# Autodesk Inventor assembly: Vise
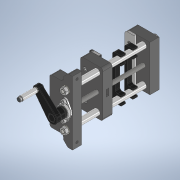
[picture p0: Inventor's stored thumbnail of the model, 180x180]
Saved by Autodesk Inventor 2020.2 (Build 242310000, 310)
## iProperties
Created: 2021-06-22
Part Number: Vise
Document SubType Name: Assembly
Designer: JK
Author: JK
## Documents named in this file (24)
- C:\Users\JK\Documents\Inventor\Vise\Vise.iam
- C:\Users\JK\Documents\Inventor\Vise\Mobile Jaw.ipt
- C:\Users\JK\Documents\Inventor\Vise\Stationary Jaw.ipt
- C:\Users\JK\Documents\Inventor\Vise\Aluminium Tube.ipt
- C:\Users\JK\Documents\Inventor\Vise\Stationary Jaw2.ipt
- C:\Users\JK\Documents\Inventor\Vise\Threaded Rod 200mm.ipt
- C:\Users\JK\Documents\Inventor\Vise\M8 Washer.ipt
- C:\Users\JK\Documents\Inventor\Vise\M8 Nut.ipt
- C:\Users\JK\Documents\Inventor\Vise\KFL08 Bearing.ipt
- C:\Users\JK\Documents\Inventor\Vise\Rubber plate.ipt
- C:\Users\JK\Documents\Inventor\Vise\Threaded Rod 210mm.ipt
- C:\Users\JK\Documents\Inventor\Vise\M5x20 Bolt.ipt
- C:\Users\JK\Documents\Inventor\Vise\M5 Low profile Nut.ipt
- C:\Users\JK\Documents\Inventor\Vise\Accessory flat surface.ipt
- C:\Users\JK\Documents\Inventor\Vise\M5 Nut.ipt
- C:\Users\JK\Documents\Inventor\Vise\Crank.ipt
- C:\Users\JK\Documents\Inventor\Vise\End-Nut.ipt
- C:\Users\JK\Documents\Inventor\Vise\M3 nut.ipt
- C:\Users\JK\Documents\Inventor\Vise\M5x50 Bolt.ipt
- C:\Users\JK\Documents\Inventor\Vise\Spacer.ipt
- C:\Users\JK\Documents\Inventor\Vise\M5 Washer.ipt
- C:\Users\JK\Documents\Inventor\Vise\M5 Lock nut.ipt
- C:\Users\JK\Documents\Inventor\Vise\RubberPiece.ipt
- C:\Users\JK\Documents\Inventor\Vise\M3x6 Set Screw.ipt
## Components (48 placed, 23 different names)
1. Mobile Jaw:1 — Mate:5, Mate:6, Mate:34, Mate:35, Mate:36, Mate:40, Mate:41, Flush:4, Angle:5, Mate:97
2. Stationary Jaw:1 — Mate:1, Mate:2, Mate:3, Mate:4, Mate:10, Mate:11, Mate:20, Mate:22, Mate:31, Mate:32, Mate:33, Mate:38, Mate:39, Flush:5, Mate:50
3. Aluminium Tube:1 — Mate:1, Mate:3, Mate:6, Mate:8, Mate:48, Mate:79
4. Aluminium Tube:2 — Mate:2, Mate:4, Mate:5, Mate:7, Mate:9, Mate:49
5. Stationary Jaw2:1 — Mate:7, Mate:8, Mate:9, Mate:25, Mate:27, Mate:28, Mate:29, Mate:30, Mate:51, Mate:52, Mate:53
6. Threaded Rod 200mm:1 — Mate:11, Mate:12, Mate:13, Mate:17, Mate:18, Flush:1
7. Threaded Rod 200mm:2 — Mate:10, Mate:14, Mate:15, Mate:16, Mate:19, Flush:2
8. M8 Washer:1 — Mate:16, Mate:20, Mate:95
9. M8 Washer:2 — Mate:12, Mate:24, Mate:25
10. M8 Washer:3 — Mate:14, Mate:26, Mate:27
11. M8 Washer:4 — Mate:17, Mate:22, Mate:23
12. M8 Nut:1 — Mate:18, Mate:23
13. M8 Nut:2 — Mate:13, Mate:24, Flush:1
14. M8 Nut:3 — Mate:15, Mate:26, Flush:2
15. M8 Nut:4 — Mate:19, Mate:95
16. KFL08 Bearing:1 — Mate:28, Mate:29, Mate:30, Mate:37, Mate:54, Mate:55, Mate:56
17. Rubber plate:1 — Mate:31, Mate:32, Mate:33, Mate:47, Mate:89, Flush:13, Mate:90
18. Rubber plate:2 — Mate:34, Mate:35, Mate:36, Mate:46, Mate:91, Mate:92, Flush:14
19. Threaded Rod 210mm:1 — Mate:37, Mate:50, Mate:72, Mate:76, Mate:96
20. M5x20 Bolt:1 — Mate:40, Flush:3, Flush:4, Mate:44
21. M5x20 Bolt:2 — Mate:39, Flush:6, Mate:42
22. M5x20 Bolt:3 — Mate:38, Flush:5, Flush:6, Mate:43
23. M5x20 Bolt:4 — Mate:41, Flush:3, Mate:45
24. M5 Low profile Nut:1 — Mate:45, Flush:7, Mate:46
25. M5 Low profile Nut:2 — Mate:42, Flush:8, Mate:47
26. M5 Low profile Nut:3 — Mate:43, Flush:8
27. M5 Low profile Nut:4 — Mate:44, Flush:7
28. Accessory flat surface:1 — Mate:48, Mate:49, Flush:11
29. M5 Nut:1 — Mate:52, Flush:9
30. M5 Nut:2 — Mate:51, Flush:9, Mate:53
31. M5x20 Bolt:5 — Mate:56, Flush:10
32. M5x20 Bolt:6 — Mate:54, Mate:55, Flush:10
33. Crank:1 — Mate:70, Mate:71, Angle:2, Mate:77, Angle:4, Mate:78, Mate:80, Mate:83, Mate:84
34. M5 Nut:3 — Mate:70, Mate:71, Angle:2
35. End-Nut:1 — Mate:72, Mate:73, Mate:74, Mate:75, Angle:3, Mate:76, Mate:77, Angle:4, Mate:78, Mate:94
36. M3 nut:1 — Mate:74, Mate:75, Angle:3, Flush:16
37. M3 nut:2 — Mate:73, Mate:93, Flush:15
38. Accessory flat surface:2 — Mate:79, Flush:11
39. M5x50 Bolt:1 — Mate:80, Mate:81, Mate:82, Mate:85, Mate:86, Mate:88, Flush:12
40. Spacer:1 — Mate:86, Mate:87
41. M5 Washer:1 — Mate:81, Mate:83, Mate:85
42. M5 Washer:2 — Mate:82, Mate:84, Mate:87
43. M5 Lock nut:1 — Mate:88, Flush:12
44. RubberPiece:1 — Mate:91, Mate:92, Flush:14
45. RubberPiece:2 — Mate:89, Flush:13, Mate:90
46. M3x6 Set Screw:1 — Mate:93, Flush:15
47. M3x6 Set Screw:2 — Mate:94, Flush:16
48. M8 Nut:5 — Mate:96, Angle:5, Mate:97
## Relationships (103: Mate 83, Flush 16, Angle 4)
- Mate:1: Stationary Jaw:1 ↔ Aluminium Tube:1
- Mate:2: Stationary Jaw:1 ↔ Aluminium Tube:2
- Mate:3: Stationary Jaw:1 ↔ Aluminium Tube:1
- Mate:4: Stationary Jaw:1 ↔ Aluminium Tube:2
- Mate:5: Mobile Jaw:1 ↔ Aluminium Tube:2
- Mate:6: Mobile Jaw:1 ↔ Aluminium Tube:1
- Mate:7: Aluminium Tube:2 ↔ Stationary Jaw2:1
- Mate:8: Aluminium Tube:1 ↔ Stationary Jaw2:1
- Mate:9: Aluminium Tube:2 ↔ Stationary Jaw2:1
- Mate:10: Stationary Jaw:1 ↔ Threaded Rod 200mm:2
- Mate:11: Stationary Jaw:1 ↔ Threaded Rod 200mm:1
- Mate:12: Threaded Rod 200mm:1 ↔ M8 Washer:2
- Mate:13: Threaded Rod 200mm:1 ↔ M8 Nut:2
- Mate:14: Threaded Rod 200mm:2 ↔ M8 Washer:3
- Mate:15: Threaded Rod 200mm:2 ↔ M8 Nut:3
- Mate:16: Threaded Rod 200mm:2 ↔ M8 Washer:1
- Mate:17: Threaded Rod 200mm:1 ↔ M8 Washer:4
- Mate:18: Threaded Rod 200mm:1 ↔ M8 Nut:1
- Mate:19: Threaded Rod 200mm:2 ↔ M8 Nut:4
- Mate:20: Stationary Jaw:1 ↔ M8 Washer:1
- Mate:22: Stationary Jaw:1 ↔ M8 Washer:4
- Mate:23: M8 Washer:4 ↔ M8 Nut:1
- Mate:24: M8 Washer:2 ↔ M8 Nut:2
- Mate:25: Stationary Jaw2:1 ↔ M8 Washer:2
- Mate:26: M8 Washer:3 ↔ M8 Nut:3
- Mate:27: Stationary Jaw2:1 ↔ M8 Washer:3
- Flush:1: Threaded Rod 200mm:1 ↔ M8 Nut:2
- Flush:2: Threaded Rod 200mm:2 ↔ M8 Nut:3
- Mate:28: Stationary Jaw2:1 ↔ KFL08 Bearing:1
- Mate:29: Stationary Jaw2:1 ↔ KFL08 Bearing:1
- Mate:30: Stationary Jaw2:1 ↔ KFL08 Bearing:1
- Mate:31: Stationary Jaw:1 ↔ Rubber plate:1
- Mate:32: Stationary Jaw:1 ↔ Rubber plate:1
- Mate:33: Stationary Jaw:1 ↔ Rubber plate:1
- Mate:34: Mobile Jaw:1 ↔ Rubber plate:2
- Mate:35: Mobile Jaw:1 ↔ Rubber plate:2
- Mate:36: Mobile Jaw:1 ↔ Rubber plate:2
- Mate:37: KFL08 Bearing:1 ↔ Threaded Rod 210mm:1
- Mate:38: Stationary Jaw:1 ↔ M5x20 Bolt:3
- Mate:39: Stationary Jaw:1 ↔ M5x20 Bolt:2
- Mate:40: Mobile Jaw:1 ↔ M5x20 Bolt:1
- Mate:41: Mobile Jaw:1 ↔ M5x20 Bolt:4
- Flush:3: M5x20 Bolt:1 ↔ M5x20 Bolt:4
- Flush:4: Mobile Jaw:1 ↔ M5x20 Bolt:1
- Flush:5: Stationary Jaw:1 ↔ M5x20 Bolt:3
- Flush:6: M5x20 Bolt:2 ↔ M5x20 Bolt:3
- Mate:42: M5x20 Bolt:2 ↔ M5 Low profile Nut:2
- Mate:43: M5x20 Bolt:3 ↔ M5 Low profile Nut:3
- Mate:44: M5x20 Bolt:1 ↔ M5 Low profile Nut:4
- Mate:45: M5x20 Bolt:4 ↔ M5 Low profile Nut:1
- Flush:7: M5 Low profile Nut:1 ↔ M5 Low profile Nut:4
- Mate:46: Rubber plate:2 ↔ M5 Low profile Nut:1
- Flush:8: M5 Low profile Nut:2 ↔ M5 Low profile Nut:3
- Mate:47: Rubber plate:1 ↔ M5 Low profile Nut:2
- Mate:48: Aluminium Tube:1 ↔ Accessory flat surface:1
- Mate:49: Aluminium Tube:2 ↔ Accessory flat surface:1
- Mate:50: Stationary Jaw:1 ↔ Threaded Rod 210mm:1
- Mate:51: Stationary Jaw2:1 ↔ M5 Nut:2
- Mate:52: Stationary Jaw2:1 ↔ M5 Nut:1
- Flush:9: M5 Nut:1 ↔ M5 Nut:2
- Mate:53: Stationary Jaw2:1 ↔ M5 Nut:2
- Mate:54: KFL08 Bearing:1 ↔ M5x20 Bolt:6
- Mate:55: KFL08 Bearing:1 ↔ M5x20 Bolt:6
- Mate:56: KFL08 Bearing:1 ↔ M5x20 Bolt:5
- Flush:10: M5x20 Bolt:5 ↔ M5x20 Bolt:6
- Mate:70: Crank:1 ↔ M5 Nut:3
- Mate:71: Crank:1 ↔ M5 Nut:3
- Angle:2 (0 deg): Crank:1 ↔ M5 Nut:3
- Mate:72: Threaded Rod 210mm:1 ↔ End-Nut:1
- Mate:73: End-Nut:1 ↔ M3 nut:2
- Mate:74: End-Nut:1 ↔ M3 nut:1
- Mate:75: End-Nut:1 ↔ M3 nut:1
- Angle:3 (0 deg): End-Nut:1 ↔ M3 nut:1
- Mate:76: Threaded Rod 210mm:1 ↔ End-Nut:1
- Mate:77: Crank:1 ↔ End-Nut:1
- Angle:4 (0 deg): Crank:1 ↔ End-Nut:1
- Mate:78: Crank:1 ↔ End-Nut:1
- Mate:79: Aluminium Tube:1 ↔ Accessory flat surface:2
- Flush:11: Accessory flat surface:1 ↔ Accessory flat surface:2
- Mate:80: Crank:1 ↔ M5x50 Bolt:1
- Mate:81: M5x50 Bolt:1 ↔ M5 Washer:1
- Mate:82: M5x50 Bolt:1 ↔ M5 Washer:2
- Mate:83: Crank:1 ↔ M5 Washer:1
- Mate:84: Crank:1 ↔ M5 Washer:2
- Mate:85: M5x50 Bolt:1 ↔ M5 Washer:1
- Mate:86: M5x50 Bolt:1 ↔ Spacer:1
- Mate:87: Spacer:1 ↔ M5 Washer:2
- Mate:88: M5x50 Bolt:1 ↔ M5 Lock nut:1
- Flush:12: M5x50 Bolt:1 ↔ M5 Lock nut:1
- Mate:89: Rubber plate:1 ↔ RubberPiece:2
- Flush:13: Rubber plate:1 ↔ RubberPiece:2
- Mate:90: Rubber plate:1 ↔ RubberPiece:2
- Mate:91: Rubber plate:2 ↔ RubberPiece:1
- Mate:92: Rubber plate:2 ↔ RubberPiece:1
- Flush:14: Rubber plate:2 ↔ RubberPiece:1
- Mate:93: M3 nut:2 ↔ M3x6 Set Screw:1
- Flush:15: M3 nut:2 ↔ M3x6 Set Screw:1
- Mate:94: End-Nut:1 ↔ M3x6 Set Screw:2
- Flush:16: M3 nut:1 ↔ M3x6 Set Screw:2
- Mate:95: M8 Washer:1 ↔ M8 Nut:4
- Mate:96: Threaded Rod 210mm:1 ↔ M8 Nut:5
- Angle:5 (0 deg): Mobile Jaw:1 ↔ M8 Nut:5
- Mate:97: Mobile Jaw:1 ↔ M8 Nut:5
